# Autodesk Inventor assembly: link_foot
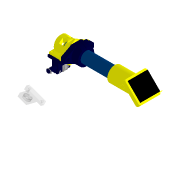
[picture p0: Inventor's stored thumbnail of the model, 180x180]
Saved by Autodesk Inventor 2020.5 (Build 245400000, 400)
## iProperties
Created: 2022-10-31
Part Number: link_foot
Document SubType Name: Assembly
Designer: Administrator
Author: Administrator
## Documents named in this file (10)
- C:\Users\Administrator\Documents\kamuy2\kamuy2\link_foot.iam
- C:\Users\Administrator\Documents\kamuy2\kamuy2\Parts\BGHK6800VV-30_Autodesk_Inventor_2020_20221102\AIS2020\BGHK6800VV-30_MIR_CPY_MIR1.iam
- C:\Users\Administrator\Documents\kamuy2\kamuy2\Parts\PIJX30-20-150_Autodesk_Inventor_2020_20221115\PIJX30-20-150_MIR_MIR_MIR1_MIR_MIR.ipt
- C:\Users\Administrator\Documents\kamuy2\kamuy2\Parts\C-SHA10_Autodesk_Inventor_2020_20221104\AIS2020\C-SHA10_MIR_MIR_MIR1_MIR_MIR.iam
- C:\Users\Administrator\Documents\kamuy2\kamuy2\Parts\HTPA30S3M060-A-N10_Autodesk_Inventor_2020_20221115\AIS2020\HTPA30S3M060-A-N10_MIR_MIR_MIR1_MIR_MIR.iam
- C:\Users\Administrator\Documents\kamuy2\kamuy2\Parts\SMYHF30_STEP_AP203AP214\SMYHF30_203_MIR_MIR_MIR1_MIR_MIR.ipt
- C:\Users\Administrator\Documents\kamuy2\kamuy2\Parts\NSFMRRA10-74-B3-S3-KC31.5-A11_Autodesk_Inventor_2020_20221116\AIS2020\NSFMRRA10-74-B3-S3-KC31_5-A11(000_000)_MIR_MIR_MIR1_MIR_MIR.iam
- C:\Users\Administrator\Documents\kamuy2\kamuy2\3dprinter\Part77_MIR.ipt
- C:\Users\Administrator\Documents\foot3d.ipt
- C:\Users\Administrator\Documents\gom.ipt
## Components (10 placed, 9 different names)
1. BGHK6800VV-30_MIR_CPY_MIR1:2 [sub-assembly]
2. PIJX30-20-150_MIR_MIR_MIR1_MIR_MIR:1 — フラッシュ:28, メイト:67
3. C-SHA10_MIR_MIR_MIR1_MIR_MIR:1 [sub-assembly] — メイト:60
4. C-SHA10_MIR_MIR_MIR1_MIR_MIR:2 [sub-assembly]
5. HTPA30S3M060-A-N10_MIR_MIR_MIR1_MIR_MIR:1 [sub-assembly] — メイト:60
6. SMYHF30_203_MIR_MIR_MIR1_MIR_MIR:1
7. NSFMRRA10-74-B3-S3-KC31_5-A11(000_000)_MIR_MIR_MIR1_MIR_MIR:1 [sub-assembly] — メイト:70
8. Part77_MIR:1 — フラッシュ:30, メイト:71
9. foot3d:1 — フラッシュ:28, フラッシュ:29, メイト:67, メイト:68, メイト:69, フラッシュ:30, フラッシュ:31
10. gom:1 — フラッシュ:29, メイト:68, メイト:69
## Relationships (23: Mate 14, Flush 9)
- [Flush]: C-SHA10_MIR_MIR_MIR1_MIR_MIR:1 ↔ C-SHA10_MIR_MIR_MIR1_MIR_MIR:2
- [Flush]: C-SHA10_MIR_MIR_MIR1_MIR_MIR:1 ↔ C-SHA10_MIR_MIR_MIR1_MIR_MIR:2
- [Mate]: C-SHA10_MIR_MIR_MIR1_MIR_MIR:2 ↔ HTPA30S3M060-A-N10_MIR_MIR_MIR1_MIR_MIR:1
- [Flush] (-20 mm): PIJX30-20-150_MIR_MIR_MIR1_MIR_MIR:1 ↔ SMYHF30_203_MIR_MIR_MIR1_MIR_MIR:1
- [Flush] (-20 mm): C-SHA10_MIR_MIR_MIR1_MIR_MIR:2 ↔ SMYHF30_203_MIR_MIR_MIR1_MIR_MIR:1
- [Mate] (15 mm): C-SHA10_MIR_MIR_MIR1_MIR_MIR:2 ↔ SMYHF30_203_MIR_MIR_MIR1_MIR_MIR:1
- [Mate]: PIJX30-20-150_MIR_MIR_MIR1_MIR_MIR:1 ↔ SMYHF30_203_MIR_MIR_MIR1_MIR_MIR:1
- [Flush] (31.5 mm): HTPA30S3M060-A-N10_MIR_MIR_MIR1_MIR_MIR:1 ↔ NSFMRRA10-74-B3-S3-KC31_5-A11(000_000)_MIR_MIR_MIR1_MIR_MIR:1
- [Mate]: C-SHA10_MIR_MIR_MIR1_MIR_MIR:1 ↔ NSFMRRA10-74-B3-S3-KC31_5-A11(000_000)_MIR_MIR_MIR1_MIR_MIR:1
- [Mate]: HTPA30S3M060-A-N10_MIR_MIR_MIR1_MIR_MIR:1 ↔ NSFMRRA10-74-B3-S3-KC31_5-A11(000_000)_MIR_MIR_MIR1_MIR_MIR:1
- [Mate]: SMYHF30_203_MIR_MIR_MIR1_MIR_MIR:1 ↔ Part77_MIR:1
- [Mate]: PIJX30-20-150_MIR_MIR_MIR1_MIR_MIR:1 ↔ Part77_MIR:1
- [Mate]: C-SHA10_MIR_MIR_MIR1_MIR_MIR:2 ↔ Part77_MIR:1
- メイト:60 [Mate]: C-SHA10_MIR_MIR_MIR1_MIR_MIR:1 ↔ HTPA30S3M060-A-N10_MIR_MIR_MIR1_MIR_MIR:1
- フラッシュ:28 [Flush]: PIJX30-20-150_MIR_MIR_MIR1_MIR_MIR:1 ↔ foot3d:1
- フラッシュ:29 [Flush]: foot3d:1 ↔ gom:1
- メイト:67 [Mate]: PIJX30-20-150_MIR_MIR_MIR1_MIR_MIR:1 ↔ foot3d:1
- メイト:68 [Mate]: foot3d:1 ↔ gom:1
- メイト:69 [Mate]: foot3d:1 ↔ gom:1
- フラッシュ:30 [Flush] (10 mm): Part77_MIR:1 ↔ foot3d:1
- メイト:70 [Mate]: NSFMRRA10-74-B3-S3-KC31_5-A11(000_000)_MIR_MIR_MIR1_MIR_MIR:1
- メイト:71 [Mate] (20 mm): Part77_MIR:1
- フラッシュ:31 [Flush]: foot3d:1
## Named parameters: d61_d48 = 0 mm, d62_d49 = 0 mm, d63_d50 = 0 mm, d70_d60 = -20 mm
